# Autodesk Inventor assembly: Subensamble_mesa
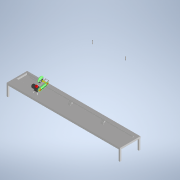
[picture p0: Inventor's stored thumbnail of the model, 180x180]
Saved by Autodesk Inventor 2021 (Build 250183000, 183)
## iProperties
Created: 2021-04-29
Part Number: Subensamble_mesa
Document SubType Name: Assembly
Designer: Admin
Author: Admin
## Documents named in this file (7)
- D:\Nelson\Documentos\Inventor\Cortadora_Automatizada\Subensamble_mesa.iam
- D:\Nelson\Documentos\Inventor\Cortadora_Automatizada\Mesa_cortadora.ipt
- D:\Nelson\Documentos\Inventor\Cortadora_Automatizada\Pata_mesa.ipt
- D:\Nelson\Documentos\Inventor\Cortadora_Automatizada\Subensamble_cortadora.iam
- D:\Nelson\Documentos\Inventor\Cortadora_Automatizada\Tubo-2_1_8.ipt
- D:\Nelson\Documentos\Inventor\Cortadora_Automatizada\Base soporte tubos.ipt
- D:\Nelson\Documentos\Inventor\Cortadora_Automatizada\193992 DSNU-32-60-PPS-A---(60PPSA---00--0-------0).iam
## Components (12 placed, 6 different names)
1. Mesa_cortadora:1 — Coincidencia:1, Coincidencia:2, Coincidencia:3, Coincidencia:4, Coincidencia:5, Coincidencia:6, Coincidencia:7, Coincidencia:8, Coincidencia:9, Coincidencia:10, Coincidencia:11, Coincidencia:12, Coincidencia:13, Coincidencia:14, Mate:15, Flush:1, Flush:2, Mate:16, Flush:3, Mate:17, Flush:4
2. Pata_mesa:1 — Coincidencia:7, Coincidencia:8, Coincidencia:9
3. Pata_mesa:2 — Coincidencia:1, Coincidencia:2, Coincidencia:3
4. Pata_mesa:3 — Coincidencia:4, Coincidencia:5, Coincidencia:6
5. Pata_mesa:4 — Coincidencia:10, Coincidencia:11, Coincidencia:12
6. Subensamble_cortadora:1 [sub-assembly] — Coincidencia:13, Coincidencia:14
7. Tubo-2_1_8:1 — Tangent:1, Tangent:2
8. Base soporte tubos:1 — Mate:15, Tangent:1, Tangent:2, Flush:1, Flush:2
9. 193992 DSNU-32-60-PPS-A---(60PPSA---00--0-------0):1 [sub-assembly]
10. 193992 DSNU-32-60-PPS-A---(60PPSA---00--0-------0):2 [sub-assembly]
11. Base soporte tubos:2 — Mate:16, Flush:3
12. Base soporte tubos:3 — Mate:17, Flush:4
## Relationships (23: Mate 17, Flush 4, Tangent 2)
- Coincidencia:1 [Mate]: Mesa_cortadora:1 ↔ Pata_mesa:2
- Coincidencia:2 [Mate]: Mesa_cortadora:1 ↔ Pata_mesa:2
- Coincidencia:3 [Mate]: Mesa_cortadora:1 ↔ Pata_mesa:2
- Coincidencia:4 [Mate]: Mesa_cortadora:1 ↔ Pata_mesa:3
- Coincidencia:5 [Mate]: Mesa_cortadora:1 ↔ Pata_mesa:3
- Coincidencia:6 [Mate]: Mesa_cortadora:1 ↔ Pata_mesa:3
- Coincidencia:7 [Mate]: Mesa_cortadora:1 ↔ Pata_mesa:1
- Coincidencia:8 [Mate]: Mesa_cortadora:1 ↔ Pata_mesa:1
- Coincidencia:9 [Mate]: Mesa_cortadora:1 ↔ Pata_mesa:1
- Coincidencia:10 [Mate]: Mesa_cortadora:1 ↔ Pata_mesa:4
- Coincidencia:11 [Mate]: Mesa_cortadora:1 ↔ Pata_mesa:4
- Coincidencia:12 [Mate]: Mesa_cortadora:1 ↔ Pata_mesa:4
- Coincidencia:13 [Mate]: Mesa_cortadora:1 ↔ Subensamble_cortadora:1
- Coincidencia:14 [Mate]: Mesa_cortadora:1 ↔ Subensamble_cortadora:1
- Mate:15: Mesa_cortadora:1 ↔ Base soporte tubos:1
- Tangent:1: Tubo-2_1_8:1 ↔ Base soporte tubos:1
- Tangent:2: Tubo-2_1_8:1 ↔ Base soporte tubos:1
- Flush:1 (297.3 mm): Mesa_cortadora:1 ↔ Base soporte tubos:1
- Flush:2 (1220 mm): Mesa_cortadora:1 ↔ Base soporte tubos:1
- Mate:16: Mesa_cortadora:1 ↔ Base soporte tubos:2
- Flush:3 (297 mm): Mesa_cortadora:1 ↔ Base soporte tubos:2
- Mate:17: Mesa_cortadora:1 ↔ Base soporte tubos:3
- Flush:4 (297 mm): Mesa_cortadora:1 ↔ Base soporte tubos:3
